# Autodesk Inventor assembly: TB_MAIN_A_001
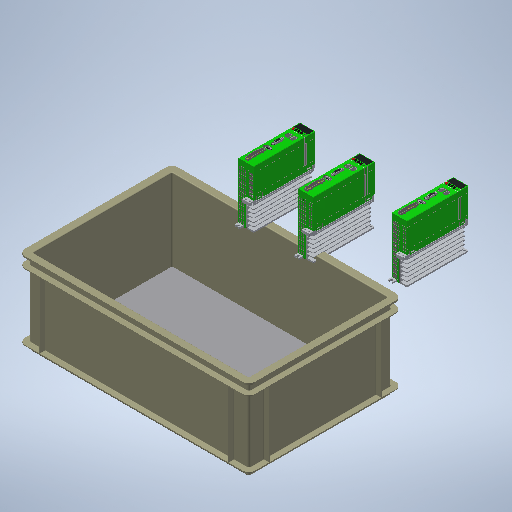
[picture p0: Inventor's stored thumbnail of the model, 512x512]
Saved by Autodesk Inventor 2025.4 (Build 294407000, 407)
## iProperties
Created: 2026-07-01
Part Number: TB_MAIN_A_001
Document SubType Name: Assembly
Designer: louis
Author: louis
## Documents named in this file (4)
- C:\Users\louis\OneDrive\Desktop\R_Trident\02_CAD\05_Top_Assembly\TB_MAIN_A_001.iam
- C:\Users\louis\OneDrive\Desktop\R_Trident\02_CAD\03_Parts_Custom\TB_FRM_MC_001_BasePlate.ipt
- C:\Users\louis\OneDrive\Desktop\R_Trident\02_CAD\01_Standard_Parts\RAKO_600x400x220_40L.ipt
- C:\Users\louis\OneDrive\Desktop\R_Trident\02_CAD\01_Standard_Parts\04_ELE_Electrical_Automation\A6-400EC\A6-400EC.iam
## Components (5 placed, 3 different names)
1. TB_FRM_MC_001_BasePlate:1 — Flush:1, Flush:2, Flush:3, Mate:1
2. RAKO_600x400x220_40L:1 — Mate:1, Mate:2, Mate:3
3. A6-400EC:1 [sub-assembly]
4. A6-400EC:2 [sub-assembly]
5. A6-400EC:3 [sub-assembly]
## Relationships (6: Flush 3, Mate 3)
- Flush:1: TB_FRM_MC_001_BasePlate:1
- Flush:2: TB_FRM_MC_001_BasePlate:1
- Flush:3: TB_FRM_MC_001_BasePlate:1
- Mate:1: TB_FRM_MC_001_BasePlate:1 ↔ RAKO_600x400x220_40L:1
- Mate:2: RAKO_600x400x220_40L:1
- Mate:3: RAKO_600x400x220_40L:1
